# Autodesk Inventor assembly: Shooter_Assembly
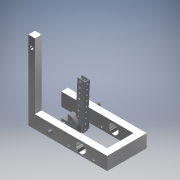
[picture p0: Inventor's stored thumbnail of the model, 180x180]
Saved by Autodesk Inventor 2019 (Build 230136000, 136)
## iProperties
Created: 2019-04-04
Part Number: Shooter_Assembly
Document SubType Name: Assembly
Designer: Delta
Author: Delta
## Documents named in this file (9)
- C:\Robotics\2019-20_CAD\offseason\random ideas\Shooter_Assembly.iam
- C:\Robotics\2019-20_CAD\offseason\random ideas\shooter.ipt
- shooter base.ipt
- C:\Robotics\2019-20_CAD\offseason\random ideas\Shooter_Stop.ipt
- C:\Robotics\COTSParts\Actobotics\585 parts\585384.ipt
- C:\Robotics\2019-20_CAD\offseason\random ideas\Shooter_Stop_Clearence.ipt
- C:\Robotics\COTSParts\Actobotics\634 parts\634064.ipt
- C:\Robotics\COTSParts\Actobotics\634 parts\634068.25inDShaft2inLong.ipt
- C:\Robotics\2019-20_CAD\offseason\random ideas\Stop.ipt
## Components (7 placed, 7 different names)
1. Shooter_Stop:1 — Insert:2, Insert:4, Insert:6
2. 585384:1 — Insert:2, Insert:3, Tangent:1
3. shooter base:1 — Insert:6
4. Shooter_Stop_Clearence:1 — Insert:3, Insert:7, Insert:8
5. 634064:1 — Insert:4, Mate:1
6. 634068.25inDShaft2inLong:1 — Insert:7, Mate:1
7. Stop:1 — Insert:8, Tangent:1
## Relationships (8: Insert 6, Mate 1, Tangent 1)
- Insert:2 (0.127 mm): Shooter_Stop:1 ↔ 585384:1
- Insert:3 (0.127 mm): 585384:1 ↔ Shooter_Stop_Clearence:1
- Insert:4: Shooter_Stop:1 ↔ 634064:1
- Insert:6 (12.7 mm): Shooter_Stop:1 ↔ shooter base:1
- Insert:7: Shooter_Stop_Clearence:1 ↔ 634068.25inDShaft2inLong:1
- Mate:1: 634064:1 ↔ 634068.25inDShaft2inLong:1
- Insert:8: Shooter_Stop_Clearence:1 ↔ Stop:1
- Tangent:1: 585384:1 ↔ Stop:1
